# Autodesk Inventor assembly: caterpillar_chain_FINAL
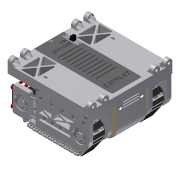
[picture p0: Inventor's stored thumbnail of the model, 180x180]
Saved by Autodesk Inventor 2015 (Build 190159000, 159)
## iProperties
Created: 2016-01-16
Part Number: caterpillar_chain_FINAL
Document SubType Name: Assembly
Designer: JavierPC
Author: JavierPC
## Documents named in this file (16)
- D:\Mis Documentos\TFM\CAD\v2\assembly\caterpillar_chain_FINAL.iam
- D:\Mis Documentos\TFM\CAD\v2\parts\platform.ipt
- D:\Mis Documentos\TFM\CAD\v2\parts\Baby GM3.ipt
- D:\Mis Documentos\TFM\CAD\v2\parts\ESP-12E DevKit.ipt
- D:\Mis Documentos\TFM\CAD\v2\parts\support_motors_1.ipt
- D:\Mis Documentos\TFM\CAD\v2\parts\Battery 7.4V.ipt
- D:\Mis Documentos\TFM\CAD\v2\parts\Electronics.ipt
- D:\Mis Documentos\TFM\CAD\v2\parts\base_lateral_cover_rigth_v2.ipt
- D:\Mis Documentos\TFM\CAD\v2\assembly\caterpillar_module_final_A.iam
- D:\Mis Documentos\TFM\CAD\v2\parts\motor_axis_cross_2.5.ipt
- C:\Users\JavierPC\Documents\Inventor\Content Center Files\R2015\es-ES\ISO 1207(1)\ISO 1207 - M2 x 12DIN EN ISO.ipt
- D:\Mis Documentos\TFM\CAD\v2\assembly\caterpillar_module_final_B.iam
- C:\Users\JavierPC\Documents\Inventor\Content Center Files\R2015\es-ES\ISO 2009(1)\ISO 2009 - M2 x 10DIN EN 8.ipt
- D:\Mis Documentos\TFM\CAD\v2\parts\platform_top_cover_v2.ipt
- C:\Users\JavierPC\Documents\Inventor\Content Center Files\R2015\es-ES\ISO 2009(1)\ISO 2009 - M2 x 12DIN EN 10.ipt
- D:\Mis Documentos\TFM\CAD\v2\parts\Switch\5MS1S102BM1QES.iam
## Components (24 placed, 15 different names)
1. platform:1 — Coincidencia:10, Coincidencia:1, Insertar:7, Insertar:8, Coincidencia:2, Ángulo:1, Coincidencia:4, Ángulo:2, Insertar:11, Coincidencia:6, Nivelación:5, Insertar:12, Nivelación:6, Coincidencia:11, Coincidencia:12, Coincidencia:13, Nivelación:7, Coincidencia:14, Coincidencia:15, Nivelación:8, Nivelación:9, Nivelación:10, Nivelación:11, Coincidencia:16, Ángulo:3, Nivelación:14, Ángulo:4, Coincidencia:19, Nivelación:15, Insertar:18, Insertar:19, Insertar:20, Insertar:21, Coincidencia:21
2. Baby GM3:1 — Coincidencia:4, Coincidencia:5, Ángulo:2, Coincidencia:18, Nivelación:13
3. motor_axis_cross_2.5:2 — Coincidencia:18, Nivelación:13
4. base_lateral_cover_rigth_v2:2 — Coincidencia:1, Coincidencia:5, Nivelación:8, Nivelación:9
5. base_lateral_cover_rigth_v2:1 — Insertar:7, Insertar:8, Coincidencia:3, Nivelación:10, Nivelación:11
6. support_motors_1:1 — Insertar:11, Coincidencia:6, Coincidencia:7, Coincidencia:8, Coincidencia:9
7. Baby GM3:2 — Coincidencia:2, Coincidencia:3, Ángulo:1, Coincidencia:17, Nivelación:12
8. motor_axis_cross_2.5:1 — Coincidencia:17, Nivelación:12
9. ESP-12E DevKit:1 — Coincidencia:7, Coincidencia:8, Coincidencia:9
10. platform_top_cover_v2:1 — Nivelación:5, Insertar:12, Nivelación:6, Insertar:22, Coincidencia:20, Coincidencia:22
11. Battery 7.4V:1 — Coincidencia:12, Coincidencia:13, Nivelación:7
12. Electronics:1 — Coincidencia:14, Coincidencia:15
13. caterpillar_module_final_A:1 [sub-assembly] — Coincidencia:16, Ángulo:3, Nivelación:14, Insertar:13, Insertar:14
14. DIN EN ISO 1207 M2 x 12:1 — Insertar:13
15. DIN EN ISO 1207 M2 x 12:2 — Insertar:16
16. DIN EN ISO 1207 M2 x 12:3 — Insertar:14
17. DIN EN ISO 1207 M2 x 12:4 — Insertar:17
18. caterpillar_module_final_B:1 [sub-assembly] — Insertar:16, Ángulo:4, Coincidencia:19, Nivelación:15, Insertar:17
19. DIN EN ISO 2009 M2 x 10:1 — Insertar:18
20. DIN EN ISO 2009 M2 x 10:2 — Insertar:19
21. DIN EN ISO 2009 M2 x 10:3 — Insertar:21
22. DIN EN ISO 2009 M2 x 10:4 — Insertar:20
23. DIN EN ISO 2009 M2 x 12:1 — Insertar:22
24. 5MS1S102BM1QES:1 [sub-assembly] — Coincidencia:20, Coincidencia:21, Coincidencia:22
## Relationships (52: Mate 22, Insert 15, Flush 11, Angle 4)
- Coincidencia:10 [Mate]: platform:1
- Coincidencia:1 [Mate]: platform:1 ↔ base_lateral_cover_rigth_v2:2
- Insertar:7: platform:1 ↔ base_lateral_cover_rigth_v2:1
- Insertar:8: platform:1 ↔ base_lateral_cover_rigth_v2:1
- [Insert]: Baby GM3:1 ↔ motor_axis_cross_2.5:2
- [Insert]: Baby GM3:2 ↔ motor_axis_cross_2.5:1
- Coincidencia:2 [Mate]: platform:1 ↔ Baby GM3:2
- Coincidencia:3 [Mate]: base_lateral_cover_rigth_v2:1 ↔ Baby GM3:2
- Ángulo:1 [Angle] (0 deg): platform:1 ↔ Baby GM3:2
- Coincidencia:4 [Mate]: platform:1 ↔ Baby GM3:1
- Coincidencia:5 [Mate]: Baby GM3:1 ↔ base_lateral_cover_rigth_v2:2
- Ángulo:2 [Angle] (180 deg): platform:1 ↔ Baby GM3:1
- Insertar:11: platform:1 ↔ support_motors_1:1
- Coincidencia:6 [Mate]: platform:1 ↔ support_motors_1:1
- Coincidencia:7 [Mate]: support_motors_1:1 ↔ ESP-12E DevKit:1
- Coincidencia:8 [Mate]: support_motors_1:1 ↔ ESP-12E DevKit:1
- Coincidencia:9 [Mate]: support_motors_1:1 ↔ ESP-12E DevKit:1
- Nivelación:5 [Flush]: platform:1 ↔ platform_top_cover_v2:1
- Insertar:12: platform:1 ↔ platform_top_cover_v2:1
- Nivelación:6 [Flush]: platform:1 ↔ platform_top_cover_v2:1
- Coincidencia:11 [Mate]: platform:1
- Coincidencia:12 [Mate]: platform:1 ↔ Battery 7.4V:1
- Coincidencia:13 [Mate]: platform:1 ↔ Battery 7.4V:1
- Nivelación:7 [Flush]: platform:1 ↔ Battery 7.4V:1
- Coincidencia:14 [Mate]: platform:1 ↔ Electronics:1
- Coincidencia:15 [Mate]: platform:1 ↔ Electronics:1
- Nivelación:8 [Flush]: platform:1 ↔ base_lateral_cover_rigth_v2:2
- Nivelación:9 [Flush]: platform:1 ↔ base_lateral_cover_rigth_v2:2
- Nivelación:10 [Flush]: platform:1 ↔ base_lateral_cover_rigth_v2:1
- Nivelación:11 [Flush]: platform:1 ↔ base_lateral_cover_rigth_v2:1
- Coincidencia:16 [Mate]: platform:1 ↔ caterpillar_module_final_A:1
- Ángulo:3 [Angle] (180 deg): platform:1 ↔ caterpillar_module_final_A:1
- Coincidencia:17 [Mate]: Baby GM3:2 ↔ motor_axis_cross_2.5:1
- Nivelación:12 [Flush]: Baby GM3:2 ↔ motor_axis_cross_2.5:1
- Coincidencia:18 [Mate]: Baby GM3:1 ↔ motor_axis_cross_2.5:2
- Nivelación:13 [Flush]: Baby GM3:1 ↔ motor_axis_cross_2.5:2
- Nivelación:14 [Flush]: platform:1 ↔ caterpillar_module_final_A:1
- Insertar:13: caterpillar_module_final_A:1 ↔ DIN EN ISO 1207 M2 x 12:1
- Insertar:14: caterpillar_module_final_A:1 ↔ DIN EN ISO 1207 M2 x 12:3
- Insertar:16: DIN EN ISO 1207 M2 x 12:2 ↔ caterpillar_module_final_B:1
- Ángulo:4 [Angle] (180 deg): platform:1 ↔ caterpillar_module_final_B:1
- Coincidencia:19 [Mate]: platform:1 ↔ caterpillar_module_final_B:1
- Nivelación:15 [Flush]: platform:1 ↔ caterpillar_module_final_B:1
- Insertar:17: DIN EN ISO 1207 M2 x 12:4 ↔ caterpillar_module_final_B:1
- Insertar:18: platform:1 ↔ DIN EN ISO 2009 M2 x 10:1
- Insertar:19: platform:1 ↔ DIN EN ISO 2009 M2 x 10:2
- Insertar:20: platform:1 ↔ DIN EN ISO 2009 M2 x 10:4
- Insertar:21: platform:1 ↔ DIN EN ISO 2009 M2 x 10:3
- Insertar:22: platform_top_cover_v2:1 ↔ DIN EN ISO 2009 M2 x 12:1
- Coincidencia:20 [Mate]: platform_top_cover_v2:1 ↔ 5MS1S102BM1QES:1
- Coincidencia:21 [Mate]: platform:1 ↔ 5MS1S102BM1QES:1
- Coincidencia:22 [Mate]: platform_top_cover_v2:1 ↔ 5MS1S102BM1QES:1
## Named parameters: d250_d249 = 0 mm
